# Autodesk Inventor assembly: FinalAssembly
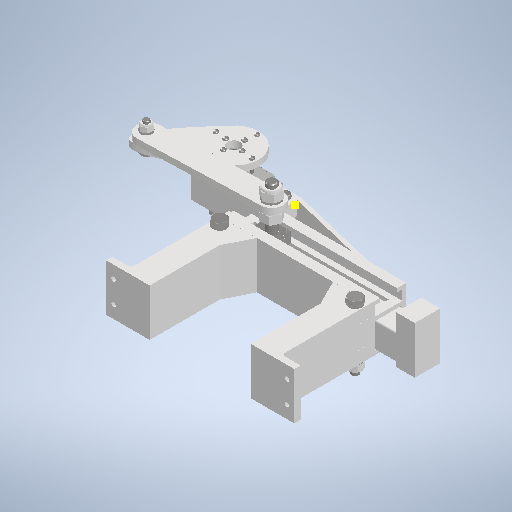
[picture p0: Inventor's stored thumbnail of the model, 512x512]
Saved by Autodesk Inventor 2025.2 (Build 292293000, 293)
## iProperties
Created: 2025-05-26
Part Number: FinalAssembly
Document SubType Name: Assembly
Designer: patrickandersen
Author: patrickandersen
## Documents named in this file (21)
- C:\Users\patrickandersen\Desktop\Linear Actuator CAD\Assembly\FinalAssembly.iam
- C:\Users\patrickandersen\Documents\shaft4V1.ipt
- C:\Users\patrickandersen\Documents\Inventor\Content Center Files\R2025\en-US\AS 1110\AS 1110 - M8 x 60.ipt
- C:\Users\patrickandersen\Downloads\90576A815_Medium-Strength Steel Nylon-Insert Locknut\90576A815_Medium-Strength Steel Nylon-Insert Locknut\90576A815_Medium-Strength Steel Nylon-Insert Locknut.ipt
- C:\Users\patrickandersen\Documents\shaftHolder4V1.ipt
- C:\Users\patrickandersen\Documents\Inventor\Content Center Files\R2025\en-US\BS 3469(2)\BS 3469 - 10 - 8 x 22 x 7.ipt
- C:\Users\patrickandersen\Downloads\Parallax-900-00005-08-25-Servo-CR-HSCR-STD\Parallax-900-00005-08-25-Servo-CR-HSCR-STD\Parallax-900-00005-08-25-Servo-CR-HSCR-STD\Parallax-900-00005-08-25-Servo-CR-HSCR-STD.ipt
- C:\Users\patrickandersen\Documents\Servo-head.finalV1.ipt
- C:\Users\patrickandersen\Documents\crankRod1.ipt
- C:\Users\patrickandersen\Documents\Inventor\Content Center Files\R2025\en-US\AS 1237 (2.1)\AS 1237 - 5.ipt
- C:\Users\patrickandersen\Downloads\90576A813_Medium-Strength Steel Nylon-Insert Locknut\90576A813_Medium-Strength Steel Nylon-Insert Locknut\90576A813_Medium-Strength Steel Nylon-Insert Locknut.ipt
- C:\Users\patrickandersen\Documents\Inventor\Content Center Files\R2025\en-US\AS 1110\AS 1110 - M5 x 20.ipt
- C:\Users\patrickandersen\Documents\Inventor\Content Center Files\R2025\en-US\AS 1237 (2.1)\AS 1237 - 8.ipt
- C:\Users\patrickandersen\Documents\legsv1.ipt
- C:\Users\patrickandersen\Documents\Inventor\Content Center Files\R2025\en-US\AS 1110\AS 1110 - M6 x 50.ipt
- C:\Users\patrickandersen\Documents\Inventor\Content Center Files\R2025\en-US\AS 1237 (2.1)\AS 1237 - 6.ipt
- C:\Users\patrickandersen\Downloads\93625A250_18-8 Stainless Steel Nylon-Insert Locknut\93625A250_18-8 Stainless Steel Nylon-Insert Locknut\93625A250_18-8 Stainless Steel Nylon-Insert Locknut.ipt
- C:\Users\patrickandersen\Documents\Inventor\Content Center Files\R2025\en-US\AS 1427(05)\AS 1427 - M4 x 16(5) II.ipt
- C:\Users\patrickandersen\Documents\Inventor\Content Center Files\R2025\en-US\AS 1237 (2.1)\AS 1237 - 4.ipt
- C:\Users\patrickandersen\Downloads\90576A812_Medium-Strength Steel Nylon-Insert Locknut\90576A812_Medium-Strength Steel Nylon-Insert Locknut\90576A812_Medium-Strength Steel Nylon-Insert Locknut.ipt
- C:\Users\patrickandersen\Documents\Inventor\Content Center Files\R2025\en-US\BS EN ISO 7045 H\EN ISO 7045 - M2 x 10 - 4.8 - H(1).ipt
## Components (47 placed, 20 different names)
1. shaft4V1:1 — Insert:1, Mate:1, Mate:2, Mate:3
2. AS 1110 - Metric M8 x 60:1 — Insert:1, Insert:2, Insert:3, Insert:11
3. 90576A815_Medium-Strength Steel Nylon-Insert Locknut:1 — Insert:2
4. shaftHolder4V1:1 — Mate:1, Mate:2, Mate:3, Mate:4, Mate:5, Mate:6, Mate:7, Mate:8, Mate:9, Mate:10, Mate:11, Mate:12, Insert:27, Insert:31, Insert:32, Insert:33, Insert:34, Insert:35, Insert:36, Insert:37
5. BS 3469 (Metric) 10 - 8 x 22 x 7:1 — Insert:3
6. Parallax-900-00005-08-25-Servo-CR-HSCR-STD:1 — Mate:4, Mate:5, Mate:6, Insert:4
7. Servo-head.finalV1:1 — Insert:4, Insert:8, Insert:9, Insert:38, Insert:39, Insert:40, Insert:41, Insert:42, Insert:43, Insert:44, Insert:45
8. crankRod1:1 — Insert:6, Insert:7, Insert:12, Insert:13
9. AS 1237 (2.1) 5:1 — Insert:7, Insert:8
10. AS 1237 (2.1) 5:2 — Insert:9, Insert:16
11. AS 1237 (2.1) 5:3 — Insert:6, Insert:17
12. AS 1237 (2.1) 8:1 — Insert:11, Insert:12, Insert:14
13. AS 1237 (2.1) 8:2 — Insert:13, Insert:15
14. 90576A815_Medium-Strength Steel Nylon-Insert Locknut:2 — Insert:15
15. 90576A815_Medium-Strength Steel Nylon-Insert Locknut:3 — Insert:14
16. AS 1110 - Metric M5 x 20:1 — Insert:16
17. 90576A813_Medium-Strength Steel Nylon-Insert Locknut:1 — Insert:17
18. legsv1:1 — Mate:7, Mate:8, Mate:9, Insert:23, Insert:24
19. legsv1:2 — Mate:10, Mate:11, Mate:12, Insert:19, Insert:20
20. AS 1110 - Metric M6 x 50:1 — Insert:22
21. AS 1237 (2.1) 6:1 — Insert:18, Insert:19
22. AS 1237 (2.1) 6:2 — Insert:22, Insert:23
23. AS 1237 (2.1) 6:3 — Insert:24, Insert:25
24. AS 1237 (2.1) 6:4 — Insert:20, Insert:21
25. AS 1110 - Metric M6 x 50:2 — Insert:18
26. 93625A250_18-8 Stainless Steel Nylon-Insert Locknut:1 — Insert:21
27. 93625A250_18-8 Stainless Steel Nylon-Insert Locknut:2 — Insert:25
28. AS 1427 H - Metric M4 x 16:1 — Insert:26
29. AS 1237 (2.1) 4:1 — Insert:26, Insert:27
30. AS 1427 H - Metric M4 x 16:2
31. AS 1237 (2.1) 4:2 — Insert:31
32. AS 1427 H - Metric M4 x 16:3
33. AS 1237 (2.1) 4:3 — Insert:32
34. AS 1427 H - Metric M4 x 16:4
35. AS 1237 (2.1) 4:4 — Insert:33
36. 90576A812_Medium-Strength Steel Nylon-Insert Locknut:1 — Insert:37
37. 90576A812_Medium-Strength Steel Nylon-Insert Locknut:2 — Insert:36
38. 90576A812_Medium-Strength Steel Nylon-Insert Locknut:3 — Insert:35
39. 90576A812_Medium-Strength Steel Nylon-Insert Locknut:4 — Insert:34
40. BS EN ISO 7045 H - Metric M2 x 10 - 4.8 - H:1 — Insert:44
41. BS EN ISO 7045 H - Metric M2 x 10 - 4.8 - H:2 — Insert:42
42. BS EN ISO 7045 H - Metric M2 x 10 - 4.8 - H:3 — Insert:45
43. BS EN ISO 7045 H - Metric M2 x 10 - 4.8 - H:4 — Insert:43
44. BS EN ISO 7045 H - Metric M2 x 10 - 4.8 - H:5 — Insert:39
45. BS EN ISO 7045 H - Metric M2 x 10 - 4.8 - H:6 — Insert:38
46. BS EN ISO 7045 H - Metric M2 x 10 - 4.8 - H:7 — Insert:41
47. BS EN ISO 7045 H - Metric M2 x 10 - 4.8 - H:8 — Insert:40
## Relationships (55: Insert 43, Mate 12)
- Insert:1: shaft4V1:1 ↔ AS 1110 - Metric M8 x 60:1
- Insert:2 (46 mm): AS 1110 - Metric M8 x 60:1 ↔ 90576A815_Medium-Strength Steel Nylon-Insert Locknut:1
- Mate:1 (0.2 mm): shaft4V1:1 ↔ shaftHolder4V1:1
- Mate:2: shaft4V1:1 ↔ shaftHolder4V1:1
- Mate:3 (0.25 mm): shaft4V1:1 ↔ shaftHolder4V1:1
- Insert:3 (40.5 mm): AS 1110 - Metric M8 x 60:1 ↔ BS 3469 (Metric) 10 - 8 x 22 x 7:1
- Mate:4: shaftHolder4V1:1 ↔ Parallax-900-00005-08-25-Servo-CR-HSCR-STD:1
- Mate:5: shaftHolder4V1:1 ↔ Parallax-900-00005-08-25-Servo-CR-HSCR-STD:1
- Mate:6 (0.6 mm): shaftHolder4V1:1 ↔ Parallax-900-00005-08-25-Servo-CR-HSCR-STD:1
- Insert:4: Parallax-900-00005-08-25-Servo-CR-HSCR-STD:1 ↔ Servo-head.finalV1:1
- Insert:6: crankRod1:1 ↔ AS 1237 (2.1) 5:3
- Insert:7: crankRod1:1 ↔ AS 1237 (2.1) 5:1
- Insert:8: Servo-head.finalV1:1 ↔ AS 1237 (2.1) 5:1
- Insert:9: Servo-head.finalV1:1 ↔ AS 1237 (2.1) 5:2
- Insert:11 (10.433 mm): AS 1110 - Metric M8 x 60:1 ↔ AS 1237 (2.1) 8:1
- Insert:12: crankRod1:1 ↔ AS 1237 (2.1) 8:1
- Insert:13: crankRod1:1 ↔ AS 1237 (2.1) 8:2
- Insert:14: AS 1237 (2.1) 8:1 ↔ 90576A815_Medium-Strength Steel Nylon-Insert Locknut:3
- Insert:15: AS 1237 (2.1) 8:2 ↔ 90576A815_Medium-Strength Steel Nylon-Insert Locknut:2
- Insert:16: AS 1237 (2.1) 5:2 ↔ AS 1110 - Metric M5 x 20:1
- Insert:17: AS 1237 (2.1) 5:3 ↔ 90576A813_Medium-Strength Steel Nylon-Insert Locknut:1
- Mate:7: shaftHolder4V1:1 ↔ legsv1:1
- Mate:8: shaftHolder4V1:1 ↔ legsv1:1
- Mate:9 (0.1 mm): shaftHolder4V1:1 ↔ legsv1:1
- Mate:10: shaftHolder4V1:1 ↔ legsv1:2
- Mate:11: shaftHolder4V1:1 ↔ legsv1:2
- Mate:12 (0.1 mm): shaftHolder4V1:1 ↔ legsv1:2
- Insert:18: AS 1237 (2.1) 6:1 ↔ AS 1110 - Metric M6 x 50:2
- Insert:19: legsv1:2 ↔ AS 1237 (2.1) 6:1
- Insert:20: legsv1:2 ↔ AS 1237 (2.1) 6:4
- Insert:21: AS 1237 (2.1) 6:4 ↔ 93625A250_18-8 Stainless Steel Nylon-Insert Locknut:1
- Insert:22: AS 1110 - Metric M6 x 50:1 ↔ AS 1237 (2.1) 6:2
- Insert:23: legsv1:1 ↔ AS 1237 (2.1) 6:2
- Insert:24: legsv1:1 ↔ AS 1237 (2.1) 6:3
- Insert:25: AS 1237 (2.1) 6:3 ↔ 93625A250_18-8 Stainless Steel Nylon-Insert Locknut:2
- Insert:26: AS 1427 H - Metric M4 x 16:1 ↔ AS 1237 (2.1) 4:1
- Insert:27 (2.5 mm): shaftHolder4V1:1 ↔ AS 1237 (2.1) 4:1
- [Insert]: AS 1427 H - Metric M4 x 16:2 ↔ AS 1237 (2.1) 4:2
- [Insert]: AS 1427 H - Metric M4 x 16:3 ↔ AS 1237 (2.1) 4:3
- [Insert]: AS 1427 H - Metric M4 x 16:4 ↔ AS 1237 (2.1) 4:4
- Insert:31 (2.5 mm): shaftHolder4V1:1 ↔ AS 1237 (2.1) 4:2
- Insert:32 (2.5 mm): shaftHolder4V1:1 ↔ AS 1237 (2.1) 4:3
- Insert:33 (2.5 mm): shaftHolder4V1:1 ↔ AS 1237 (2.1) 4:4
- Insert:34: shaftHolder4V1:1 ↔ 90576A812_Medium-Strength Steel Nylon-Insert Locknut:4
- Insert:35: shaftHolder4V1:1 ↔ 90576A812_Medium-Strength Steel Nylon-Insert Locknut:3
- Insert:36: shaftHolder4V1:1 ↔ 90576A812_Medium-Strength Steel Nylon-Insert Locknut:2
- Insert:37: shaftHolder4V1:1 ↔ 90576A812_Medium-Strength Steel Nylon-Insert Locknut:1
- Insert:38: Servo-head.finalV1:1 ↔ BS EN ISO 7045 H - Metric M2 x 10 - 4.8 - H:6
- Insert:39: Servo-head.finalV1:1 ↔ BS EN ISO 7045 H - Metric M2 x 10 - 4.8 - H:5
- Insert:40: Servo-head.finalV1:1 ↔ BS EN ISO 7045 H - Metric M2 x 10 - 4.8 - H:8
- Insert:41: Servo-head.finalV1:1 ↔ BS EN ISO 7045 H - Metric M2 x 10 - 4.8 - H:7
- Insert:42: Servo-head.finalV1:1 ↔ BS EN ISO 7045 H - Metric M2 x 10 - 4.8 - H:2
- Insert:43: Servo-head.finalV1:1 ↔ BS EN ISO 7045 H - Metric M2 x 10 - 4.8 - H:4
- Insert:44: Servo-head.finalV1:1 ↔ BS EN ISO 7045 H - Metric M2 x 10 - 4.8 - H:1
- Insert:45: Servo-head.finalV1:1 ↔ BS EN ISO 7045 H - Metric M2 x 10 - 4.8 - H:3
## Named parameters: d46_d44 = 0 mm, d47_d44 = 0 mm, d48_d44 = 0 mm
